# Autodesk Inventor assembly: segment3
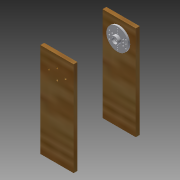
[picture p0: Inventor's stored thumbnail of the model, 180x180]
Saved by Autodesk Inventor 2013 (Build 170138000, 138)
## iProperties
Created: 2014-10-12
Part Number: segment3
Document SubType Name: Assembly
Designer: Masta
Author: Masta
## Documents named in this file (3)
- D:\DrOctopus\3D model\arm\segment3.iam
- D:\DrOctopus\3D model\arm\servo arm DS939HV round.ipt
- D:\DrOctopus\3D model\arm\segment3a.ipt
## Components (3 placed, 2 different names)
1. servo arm DS939HV round:1 — Insert:1, Insert:2
2. segment3a:1 — Insert:1, Insert:2, Mate:1, Flush:1, Flush:2
3. segment3a:2 — Mate:1, Flush:1, Flush:2
## Relationships (5: Insert 2, Flush 2, Mate 1)
- Insert:1: servo arm DS939HV round:1 ↔ segment3a:1
- Insert:2: servo arm DS939HV round:1 ↔ segment3a:1
- Mate:1 (52.6 mm): segment3a:1 ↔ segment3a:2
- Flush:1: segment3a:1 ↔ segment3a:2
- Flush:2: segment3a:1 ↔ segment3a:2
